# Autodesk Inventor assembly: sch40conduit
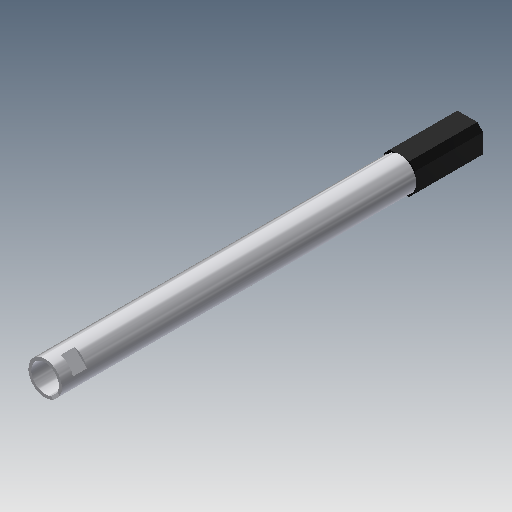
[picture p0: Inventor's stored thumbnail of the model, 512x512]
Saved by Autodesk Inventor 2019.3 (Build 233278000, 278)
## iProperties
Created: 2018-11-30
Part Number: sch40conduit
Document SubType Name: Assembly
Designer: ddeboer
Author: ddeboer
## Documents named in this file (3)
- C:\Users\Kathryn Rosie\Google Drive\HERA\Feed\CAD\Dave Conduit 20190117\sch40_conduit-master\outer_assy.iam
- C:\Users\Kathryn Rosie\Google Drive\HERA\Feed\CAD\Dave Conduit 20190117\sch40_conduit-master\conduit_endcap.ipt
- C:\Users\Kathryn Rosie\Google Drive\HERA\Feed\CAD\Dave Conduit 20190117\sch40_conduit-master\outer_sheath.ipt
## Components (2 placed, 2 different names)
1. conduit_endcap:1 — Insert:1, Angle:1
2. outer_sheath:1 — Insert:1, Angle:1
## Relationships (2: Insert 1, Angle 1)
- Insert:1 (-15 mm): conduit_endcap:1 ↔ outer_sheath:1
- Angle:1 (0 deg): conduit_endcap:1 ↔ outer_sheath:1
